# Autodesk Inventor assembly: axis3
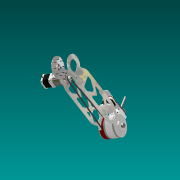
[picture p0: Inventor's stored thumbnail of the model, 180x180]
Saved by Autodesk Inventor 2020.3 (Build 243373000, 373)
## iProperties
Created: 2020-05-24
Part Number: axis3
Document SubType Name: Assembly
Designer: Svend
Author: Svend
## Documents named in this file (23)
- C:\Users\Svend\OneDrive\Documents\GitHub\BeerMinder\3D-model\axis3\axis3.iam
- C:\Users\Svend\OneDrive\Documents\GitHub\BeerMinder\3D-model\subAssembly\Nema17MetGearbox.iam
- C:\Users\Svend\OneDrive\Documents\GitHub\BeerMinder\3D-model\pulleys\GT2 Timing Pulley 20T - 8mm as.ipt
- C:\Users\Svend\OneDrive\Documents\GitHub\BeerMinder\3D-model\pulleys\Tandriem20naar60T-696mm.ipt
- C:\Users\Svend\OneDrive\Documents\GitHub\BeerMinder\3D-model\Base (Axis 1)\spiebaanBevestiging.ipt
- C:\Users\Svend\OneDrive\Documents\GitHub\BeerMinder\3D-model\pulleys\GT2 Timing Pulley 60T - 8mm as.ipt
- C:\Users\Svend\OneDrive\Documents\GitHub\BeerMinder\3D-model\bearings\Ball Bearing 608ZZ.ipt
- C:\Users\Svend\OneDrive\Documents\GitHub\BeerMinder\3D-model\Base (Axis 1)\asArm2.ipt
- C:\Users\Svend\OneDrive\Documents\GitHub\BeerMinder\3D-model\Base (Axis 1)\arm1v2.ipt
- C:\Users\Svend\OneDrive\Documents\GitHub\BeerMinder\3D-model\Base (Axis 1)\60mmspacer.ipt
- C:\Users\Svend\OneDrive\Documents\GitHub\BeerMinder\3D-model\Base (Axis 1)\60mmspacerDicht.ipt
- C:\Users\Svend\OneDrive\Documents\GitHub\BeerMinder\3D-model\bearings\stelring - 8mm.ipt
- C:\Users\Svend\OneDrive\Documents\GitHub\BeerMinder\3D-model\axis4\spacerVoorLager.ipt
- C:\Users\Svend\OneDrive\Documents\GitHub\BeerMinder\3D-model\boutjesEnMoertjes\ISO 4762 - M3 x 10ISO.ipt
- C:\Users\Svend\OneDrive\Documents\GitHub\BeerMinder\3D-model\boutjesEnMoertjes\ISO 7089 - 3 - 140 HV(1).ipt
- C:\Users\Svend\OneDrive\Documents\GitHub\BeerMinder\3D-model\boutjesEnMoertjes\ISO 10642 - M3x12.ipt
- C:\Users\Svend\OneDrive\Documents\GitHub\BeerMinder\3D-model\boutjesEnMoertjes\ISO 4035 - M3 - ISO.ipt
- C:\Users\Svend\OneDrive\Documents\GitHub\BeerMinder\3D-model\boutjesEnMoertjes\ISO 7089 - 4 - 140 HV(1).ipt
- C:\Users\Svend\OneDrive\Documents\GitHub\BeerMinder\3D-model\Base (Axis 1)\spiebaanplaatKlein.ipt
- C:\Users\Svend\OneDrive\Documents\GitHub\BeerMinder\3D-model\boutjesEnMoertjes\ISO 7380-1 - M4 x 16.ipt
- C:\Users\Svend\OneDrive\Documents\GitHub\BeerMinder\3D-model\boutjesEnMoertjes\ISO 7380-1 - M3 x 10.ipt
- C:\Users\Svend\OneDrive\Documents\GitHub\BeerMinder\3D-model\Base (Axis 1)\arm1 tweede kant.ipt
- C:\Users\Svend\OneDrive\Documents\GitHub\BeerMinder\3D-model\axis4\axis4.iam
## Components (56 placed, 22 different names)
1. Nema17MetGearbox:1 [sub-assembly] — Mate:9, Mate:33, Mate:34, Mate:35, Mate:41
2. GT2 Timing Pulley 20T - 8mm as:1 — Mate:9, Mate:91, Mate:92
3. Tandriem20naar60T-696mm:1 — Mate:91, Mate:92
4. spiebaanBevestiging:1 — Flush:4
5. GT2 Timing Pulley 60T - 8mm as:1
6. Ball Bearing 608ZZ:1
7. asArm2:1 — Mate:89, Mate:94, Mate:98, Mate:100
8. arm1v2:1 — Mate:22, Mate:23, Mate:36, Mate:37, Mate:38, Mate:39, Mate:40, Mate:43, Mate:45, Mate:59, Insert:3, Insert:4, Insert:5, Insert:6, Insert:7, Insert:8, Insert:9, Insert:10, Mate:69, Mate:76, Insert:42, Insert:43, Insert:44, Insert:45, Insert:46, Insert:47, Insert:48, Insert:49, Mate:95, Mate:97
9. 60mmspacer:1
10. 60mmspacerDicht:1 — Mate:47, Mate:49, Mate:51, Mate:53, Mate:103, Mate:104
11. stelring - 8mm:1 — Mate:102
12. spacerVoorLager:1 — Mate:22, Mate:23, Mate:59, Mate:101
13. spiebaanplaatKlein:1 — Mate:69, Flush:4, Mate:70, Mate:71, Mate:72, Mate:73, Mate:74, Mate:75, Mate:76
14. 60mmspacerDicht:2 — Mate:85, Mate:86, Mate:88, Mate:90, Mate:100
15. 60mmspacer:2 — Mate:85, Mate:86, Mate:87, Mate:98, Mate:99
16. Ball Bearing 608ZZ:2 — Mate:87, Mate:88
17. stelring - 8mm:2 — Mate:89, Mate:90
18. arm1 tweede kant:1 — Mate:94, Mate:95, Mate:97, Mate:99
19. axis4:1 [sub-assembly] — Mate:101, Mate:102
20. ISO 7380-1 M3 x 10:1 — Insert:42
21. ISO 7380-1 M3 x 10:2 — Insert:43
22. ISO 7380-1 M3 x 10:3 — Insert:44
23. ISO 7380-1 M3 x 10:4 — Insert:45
24. ISO 7380-1 M3 x 10:5 — Insert:46
25. ISO 7380-1 M3 x 10:6 — Insert:47
26. ISO 7380-1 M3 x 10:7 — Insert:48
27. ISO 7380-1 M3 x 10:8 — Insert:49
28. ISO 7380-1 M4 x 16:1 — Mate:70, Mate:71
29. ISO 7380-1 M4 x 16:3 — Mate:72, Mate:73
30. ISO 7380-1 M4 x 16:2 — Mate:74, Mate:75
31. ISO 4762 M3 x 10:1 — Mate:29, Mate:30, Mate:34
32. ISO 4762 M3 x 10:2 — Mate:25, Mate:26, Mate:35
33. ISO 4762 M3 x 10:3 — Mate:27, Mate:28, Mate:41
34. ISO 4762 M3 x 10:4 — Mate:31, Mate:32, Mate:33
35. ISO 7089 3:1 — Mate:25, Mate:26, Mate:36
36. ISO 7089 3:2 — Mate:27, Mate:28, Mate:37, Mate:38
37. ISO 7089 3:3 — Mate:29, Mate:30, Mate:39
38. ISO 7089 3:4 — Mate:31, Mate:32, Mate:40
39. ISO 10642 M3x12:2 — Mate:43, Mate:46, Mate:54
40. ISO 10642 M3x12:4 — Mate:45, Mate:52, Mate:56
41. ISO 7089 3:5 — Mate:46, Mate:47, Mate:55
42. ISO 7089 3:6 — Mate:49, Insert:1
43. ISO 7089 3:7 — Mate:51, Insert:2
44. ISO 7089 3:8 — Mate:52, Mate:53, Mate:57
45. ISO 4035 M3:1 — Mate:54, Mate:55
46. ISO 4035 M3:2 — Mate:56, Mate:57
47. ISO 4035 M3:3 — Insert:1, Mate:104
48. ISO 4035 M3:4 — Insert:2, Mate:103
49. ISO 7089 4:1 — Insert:3
50. ISO 7089 4:2 — Insert:4
51. ISO 7089 4:3 — Insert:5
52. ISO 7089 4:4 — Insert:6
53. ISO 7089 4:5 — Insert:7
54. ISO 7089 4:6 — Insert:8
55. ISO 7089 4:7 — Insert:9
56. ISO 7089 4:8 — Insert:10
## Relationships (100: Mate 77, Insert 18, Flush 4, Angle 1)
- [Mate]: Tandriem20naar60T-696mm:1 ↔ GT2 Timing Pulley 60T - 8mm as:1
- [Mate] (0.5 mm): Tandriem20naar60T-696mm:1 ↔ GT2 Timing Pulley 60T - 8mm as:1
- [Mate]: GT2 Timing Pulley 60T - 8mm as:1 ↔ Ball Bearing 608ZZ:1
- [Mate]: GT2 Timing Pulley 60T - 8mm as:1 ↔ Ball Bearing 608ZZ:1
- [Mate]: Ball Bearing 608ZZ:1 ↔ asArm2:1
- [Mate]: spiebaanBevestiging:1 ↔ arm1v2:1
- [Flush]: spiebaanBevestiging:1 ↔ arm1v2:1
- [Mate]: Nema17MetGearbox:1 ↔ arm1v2:1
- [Angle] (180 deg): Nema17MetGearbox:1 ↔ arm1v2:1
- Mate:9: Nema17MetGearbox:1 ↔ GT2 Timing Pulley 20T - 8mm as:1
- [Mate]: Nema17MetGearbox:1 ↔ arm1v2:1
- [Mate]: arm1v2:1 ↔ 60mmspacer:1
- [Mate]: arm1v2:1 ↔ 60mmspacer:1
- [Mate]: arm1v2:1 ↔ 60mmspacer:1
- [Flush]: Ball Bearing 608ZZ:1 ↔ 60mmspacer:1
- [Mate]: 60mmspacer:1 ↔ 60mmspacerDicht:1
- [Mate]: 60mmspacer:1 ↔ 60mmspacerDicht:1
- [Mate]: 60mmspacer:1 ↔ 60mmspacerDicht:1
- [Mate]: asArm2:1 ↔ stelring - 8mm:1
- [Mate]: 60mmspacerDicht:1 ↔ stelring - 8mm:1
- [Flush]: asArm2:1 ↔ stelring - 8mm:1
- [Mate]: arm1v2:1 ↔ stelring - 8mm:1
- [Mate]: spiebaanBevestiging:1 ↔ arm1v2:1
- Mate:22: arm1v2:1 ↔ spacerVoorLager:1
- Mate:23: arm1v2:1 ↔ spacerVoorLager:1
- Mate:25: ISO 4762 M3 x 10:2 ↔ ISO 7089 3:1
- Mate:26: ISO 4762 M3 x 10:2 ↔ ISO 7089 3:1
- Mate:27: ISO 4762 M3 x 10:3 ↔ ISO 7089 3:2
- Mate:28: ISO 4762 M3 x 10:3 ↔ ISO 7089 3:2
- Mate:29: ISO 4762 M3 x 10:1 ↔ ISO 7089 3:3
- Mate:30: ISO 4762 M3 x 10:1 ↔ ISO 7089 3:3
- Mate:31: ISO 4762 M3 x 10:4 ↔ ISO 7089 3:4
- Mate:32: ISO 4762 M3 x 10:4 ↔ ISO 7089 3:4
- Mate:33: Nema17MetGearbox:1 ↔ ISO 4762 M3 x 10:4
- Mate:34: Nema17MetGearbox:1 ↔ ISO 4762 M3 x 10:1
- Mate:35: Nema17MetGearbox:1 ↔ ISO 4762 M3 x 10:2
- Mate:36: arm1v2:1 ↔ ISO 7089 3:1
- Mate:37: arm1v2:1 ↔ ISO 7089 3:2
- Mate:38: arm1v2:1 ↔ ISO 7089 3:2
- Mate:39: arm1v2:1 ↔ ISO 7089 3:3
- Mate:40: arm1v2:1 ↔ ISO 7089 3:4
- Mate:41: Nema17MetGearbox:1 ↔ ISO 4762 M3 x 10:3
- Mate:43: arm1v2:1 ↔ ISO 10642 M3x12:2
- Mate:45: arm1v2:1 ↔ ISO 10642 M3x12:4
- Mate:46: ISO 10642 M3x12:2 ↔ ISO 7089 3:5
- Mate:47: 60mmspacerDicht:1 ↔ ISO 7089 3:5
- Mate:49: 60mmspacerDicht:1 ↔ ISO 7089 3:6
- Mate:51: 60mmspacerDicht:1 ↔ ISO 7089 3:7
- Mate:52: ISO 10642 M3x12:4 ↔ ISO 7089 3:8
- Mate:53: 60mmspacerDicht:1 ↔ ISO 7089 3:8
- Mate:54: ISO 10642 M3x12:2 ↔ ISO 4035 M3:1
- Mate:55: ISO 7089 3:5 ↔ ISO 4035 M3:1
- Mate:56: ISO 10642 M3x12:4 ↔ ISO 4035 M3:2
- Mate:57: ISO 7089 3:8 ↔ ISO 4035 M3:2
- Insert:1: ISO 7089 3:6 ↔ ISO 4035 M3:3
- Insert:2: ISO 7089 3:7 ↔ ISO 4035 M3:4
- Mate:59: arm1v2:1 ↔ spacerVoorLager:1
- Insert:3: arm1v2:1 ↔ ISO 7089 4:1
- Insert:4: arm1v2:1 ↔ ISO 7089 4:2
- Insert:5: arm1v2:1 ↔ ISO 7089 4:3
- Insert:6: arm1v2:1 ↔ ISO 7089 4:4
- Insert:7: arm1v2:1 ↔ ISO 7089 4:5
- Insert:8: arm1v2:1 ↔ ISO 7089 4:6
- Insert:9: arm1v2:1 ↔ ISO 7089 4:7
- Insert:10: arm1v2:1 ↔ ISO 7089 4:8
- Mate:69: arm1v2:1 ↔ spiebaanplaatKlein:1
- Flush:4: spiebaanBevestiging:1 ↔ spiebaanplaatKlein:1
- Mate:70: spiebaanplaatKlein:1 ↔ ISO 7380-1 M4 x 16:1
- Mate:71: spiebaanplaatKlein:1 ↔ ISO 7380-1 M4 x 16:1
- Mate:72: spiebaanplaatKlein:1 ↔ ISO 7380-1 M4 x 16:3
- Mate:73: spiebaanplaatKlein:1 ↔ ISO 7380-1 M4 x 16:3
- Mate:74: spiebaanplaatKlein:1 ↔ ISO 7380-1 M4 x 16:2
- Mate:75: spiebaanplaatKlein:1 ↔ ISO 7380-1 M4 x 16:2
- Mate:76: arm1v2:1 ↔ spiebaanplaatKlein:1
- Insert:42: arm1v2:1 ↔ ISO 7380-1 M3 x 10:1
- Insert:43: arm1v2:1 ↔ ISO 7380-1 M3 x 10:2
- Insert:44: arm1v2:1 ↔ ISO 7380-1 M3 x 10:3
- Insert:45: arm1v2:1 ↔ ISO 7380-1 M3 x 10:4
- Insert:46: arm1v2:1 ↔ ISO 7380-1 M3 x 10:5
- Insert:47: arm1v2:1 ↔ ISO 7380-1 M3 x 10:6
- Insert:48: arm1v2:1 ↔ ISO 7380-1 M3 x 10:7
- Insert:49: arm1v2:1 ↔ ISO 7380-1 M3 x 10:8
- Mate:85: 60mmspacerDicht:2 ↔ 60mmspacer:2
- Mate:86: 60mmspacerDicht:2 ↔ 60mmspacer:2
- Mate:87: 60mmspacer:2 ↔ Ball Bearing 608ZZ:2
- Mate:88: 60mmspacerDicht:2 ↔ Ball Bearing 608ZZ:2
- Mate:89: asArm2:1 ↔ stelring - 8mm:2
- Mate:90: 60mmspacerDicht:2 ↔ stelring - 8mm:2
- Mate:91: GT2 Timing Pulley 20T - 8mm as:1 ↔ Tandriem20naar60T-696mm:1
- Mate:92 (0.5 mm): GT2 Timing Pulley 20T - 8mm as:1 ↔ Tandriem20naar60T-696mm:1
- Mate:94: asArm2:1 ↔ arm1 tweede kant:1
- Mate:95: arm1v2:1 ↔ arm1 tweede kant:1
- Mate:97 (60.6 mm): arm1v2:1 ↔ arm1 tweede kant:1
- Mate:98: asArm2:1 ↔ 60mmspacer:2
- Mate:99: 60mmspacer:2 ↔ arm1 tweede kant:1
- Mate:100: asArm2:1 ↔ 60mmspacerDicht:2
- Mate:101: spacerVoorLager:1 ↔ axis4:1
- Mate:102: stelring - 8mm:1 ↔ axis4:1
- Mate:103: 60mmspacerDicht:1 ↔ ISO 4035 M3:4
- Mate:104: 60mmspacerDicht:1 ↔ ISO 4035 M3:3
